# Autodesk Inventor assembly: Сборка2
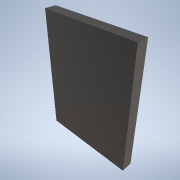
[picture p0: Inventor's stored thumbnail of the model, 180x180]
Saved by Autodesk Inventor 2020 (Build 240168000, 168)
## iProperties
Created: 2024-01-28
Part Number: Сборка2
Document SubType Name: Assembly
Designer: 4s
Author: 4s
## Documents named in this file (5)
- C:\Users\4s\Documents\Inventor models\Asterisk\Сборка2.iam
- C:\Users\4s\Documents\Inventor models\Asterisk\field.ipt
- C:\Users\4s\Documents\Inventor models\Asterisk\robot001\Asterisk_main.iam
- C:\Users\4s\Documents\Asterisk\Main board 3d\main.iam
- C:\Users\4s\Documents\Altium projects\Asterisk TSOP Board\TSOP board 3d\tsop_board_black.iam
## Components (4 placed, 4 different names)
1. field:1 — Заподлицо:1, Совмещение:1, Совмещение:2, Совмещение:3
2. Asterisk_main:1 [sub-assembly] — Совмещение:3, Совмещение:4, Совмещение:5, Совмещение:6, Совмещение:7, Угол:1, Совмещение:8
3. main:1 [sub-assembly] — Совмещение:4, Совмещение:5, Совмещение:6
4. tsop_board_black:1 [sub-assembly] — Совмещение:7, Угол:1, Совмещение:8
## Relationships (10: Mate 8, Flush 1, Angle 1)
- Заподлицо:1 [Flush]: field:1
- Совмещение:1 [Mate]: field:1
- Совмещение:2 [Mate]: field:1
- Совмещение:3 [Mate] (9.5 mm): field:1 ↔ Asterisk_main:1
- Совмещение:4 [Mate]: Asterisk_main:1 ↔ main:1
- Совмещение:5 [Mate]: Asterisk_main:1 ↔ main:1
- Совмещение:6 [Mate]: Asterisk_main:1 ↔ main:1
- Совмещение:7 [Mate]: Asterisk_main:1 ↔ tsop_board_black:1
- Угол:1 [Angle] (0 deg): Asterisk_main:1 ↔ tsop_board_black:1
- Совмещение:8 [Mate]: Asterisk_main:1 ↔ tsop_board_black:1
